# Autodesk Inventor assembly: Outer Frame 26 x 26
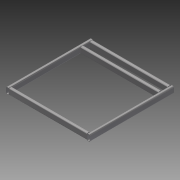
[picture p0: Inventor's stored thumbnail of the model, 180x180]
Saved by Autodesk Inventor 2015 (Build 190159000, 159)
## iProperties
Created: 2015-01-08
Part Number: Outer Frame 26 x 26
Document SubType Name: Assembly
Designer: jhirshland1
_SolveAssemblyDoc: Frame Generator Solve Assembly
_Version: 15.0.0
Author: jhirshland1
## Documents named in this file (5)
- \\internal\studentdata\HomeDir\jhirshland1\Documents\Inventor\HWRobot2015\Frame\Outer Frame 26 x 26.iam
- \\internal\studentdata\HomeDir\jhirshland1\Documents\Inventor\HWRobot2015\Frame\Frame Outline.ipt
- \\internal\studentdata\HomeDir\jhirshland1\Documents\Inventor\Assembly1\Frame\Aluminum Frame.iam
- \\internal\studentdata\HomeDir\jhirshland1\Documents\Inventor\HWRobot2015\Frame\Contact Bar for Lift.ipt
- \\internal\studentdata\HomeDir\jhirshland1\Documents\Inventor\HWRobot2015\Frame\AISC HSS - 2x1x1_8 - 15.ipt
## Components (4 placed, 4 different names)
1. Frame Outline:1
2. Aluminum Frame:1 [sub-assembly] — Flush:1, Mate:1, Mate:2
3. Contact Bar for Lift:1
4. AISC HSS - 2x1x1_8 - 15:1 — Flush:1, Mate:1, Mate:2
## Relationships (3: Mate 2, Flush 1)
- Flush:1: Aluminum Frame:1 ↔ AISC HSS - 2x1x1_8 - 15:1
- Mate:1: Aluminum Frame:1 ↔ AISC HSS - 2x1x1_8 - 15:1
- Mate:2 (50.8 mm): Aluminum Frame:1 ↔ AISC HSS - 2x1x1_8 - 15:1
